# Autodesk Inventor assembly: Assembly1
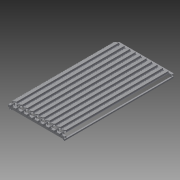
[picture p0: Inventor's stored thumbnail of the model, 180x180]
Saved by Autodesk Inventor 2015 SP1 (Build 190203100, 203)
## iProperties
Created: 2015-03-28
Part Number: Assembly1
Document SubType Name: Assembly
Designer: Cyril
Mass: 10678.5 g
Surface Area: 59183.2 cm^2
Volume: 10678.5 cm^3
Density: 1 g/cm^3
Author: Cyril
## Documents named in this file (9)
- C:\Users\Cyril\Documents\OSE FR\Concentrateur solaire\Assemblage_global.iam
- C:\Users\Cyril\Documents\OSE FR\Concentrateur solaire\Part4.ipt
- C:\Users\Cyril\Documents\OSE FR\Concentrateur solaire\Assemblage_mirroir.iam
- C:\Users\Cyril\Documents\OSE FR\Concentrateur solaire\Moteur.ipt
- C:\Users\Cyril\Documents\OSE FR\Concentrateur solaire\Accouplement.ipt
- C:\Users\Cyril\Documents\OSE FR\Concentrateur solaire\michaud_chailly_C2_151_8_128.ipt
- C:\Users\Cyril\Documents\OSE FR\Concentrateur solaire\Plaque support.ipt
- C:\Users\Cyril\Documents\OSE FR\Concentrateur solaire\Assemblage_Cadre.iam
- C:\Users\Cyril\Documents\OSE FR\Concentrateur solaire\Capteur optique.ipt
## Components (71 placed, 8 different names)
1. Assemblage_Cadre:1 [sub-assembly] — Mate:1, Flush:31, Flush:32, Mate:2, Flush:33
2. Moteur:1 — Insert:19, Insert:23, Insert:24
3. Part4:1 — Insert:23, Mate:1, Flush:31, Insert:24
4. Plaque support:1 — Insert:21, Flush:32, Mate:2, Flush:33, Insert:25, Mate:4
5. Assemblage_mirroir:3 [sub-assembly] — Insert:20, Mate:3
6. michaud_chailly_C2_151_8_128:1 — Insert:21, Mate:3
7. Accouplement:1 — Insert:19, Insert:20
8. Capteur optique:1 — Insert:25, Mate:4
9. Moteur:2
10. Part4:2
11. Plaque support:3
12. Assemblage_mirroir:4 [sub-assembly]
13. michaud_chailly_C2_151_8_128:2
14. Accouplement:2
15. Capteur optique:2
16. Moteur:3
17. Part4:3
18. Plaque support:4
19. Assemblage_mirroir:5 [sub-assembly]
20. michaud_chailly_C2_151_8_128:3
21. Accouplement:3
22. Capteur optique:3
23. Moteur:4
24. Part4:4
25. Plaque support:5
26. Assemblage_mirroir:6 [sub-assembly]
27. michaud_chailly_C2_151_8_128:4
28. Accouplement:4
29. Capteur optique:4
30. Moteur:5
31. Part4:5
32. Plaque support:6
33. Assemblage_mirroir:7 [sub-assembly]
34. michaud_chailly_C2_151_8_128:5
35. Accouplement:5
36. Capteur optique:5
37. Moteur:6
38. Part4:6
39. Plaque support:7
40. Assemblage_mirroir:8 [sub-assembly]
41. michaud_chailly_C2_151_8_128:6
42. Accouplement:6
43. Capteur optique:6
44. Moteur:7
45. Part4:7
46. Plaque support:8
47. Assemblage_mirroir:9 [sub-assembly]
48. michaud_chailly_C2_151_8_128:7
49. Accouplement:7
50. Capteur optique:7
51. Moteur:8
52. Part4:8
53. Plaque support:9
54. Assemblage_mirroir:10 [sub-assembly]
55. michaud_chailly_C2_151_8_128:8
56. Accouplement:8
57. Capteur optique:8
58. Moteur:9
59. Part4:9
60. Plaque support:10
61. Assemblage_mirroir:11 [sub-assembly]
62. michaud_chailly_C2_151_8_128:9
63. Accouplement:9
64. Capteur optique:9
65. Moteur:10
66. Part4:10
67. Plaque support:11
68. Assemblage_mirroir:12 [sub-assembly]
69. michaud_chailly_C2_151_8_128:10
70. Accouplement:10
71. Capteur optique:10
## Component patterns: (10 elements, first: Moteur:1 + Part4:1 + Plaque support:1 + Assemblage_mirroir:3 + michaud_chailly_C2_151_8_128:1 + Accouplement:1 + Capteur optique:1)
## Relationships (13: Insert 6, Mate 4, Flush 3)
- Insert:19 (-10 mm): Moteur:1 ↔ Accouplement:1
- Insert:20 (-10 mm): Assemblage_mirroir:3 ↔ Accouplement:1
- Insert:21: Plaque support:1 ↔ michaud_chailly_C2_151_8_128:1
- Insert:23: Moteur:1 ↔ Part4:1
- Mate:1: Assemblage_Cadre:1 ↔ Part4:1
- Flush:31: Assemblage_Cadre:1 ↔ Part4:1
- Flush:32 (-43 mm): Assemblage_Cadre:1 ↔ Plaque support:1
- Insert:24: Moteur:1 ↔ Part4:1
- Mate:2: Assemblage_Cadre:1 ↔ Plaque support:1
- Flush:33 (18.5 mm): Assemblage_Cadre:1 ↔ Plaque support:1
- Mate:3: Assemblage_mirroir:3 ↔ michaud_chailly_C2_151_8_128:1
- Insert:25: Plaque support:1 ↔ Capteur optique:1
- Mate:4: Plaque support:1 ↔ Capteur optique:1
